# Autodesk Inventor assembly: Assembly_Cube_Kinematic_Mirrormount_Thorlabs_45_PRO_v3
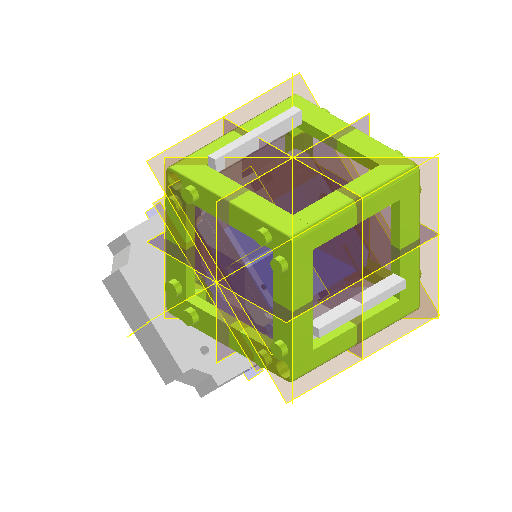
[picture p0: Inventor's stored thumbnail of the model, 512x512]
Saved by Autodesk Inventor 2022 (Build 260153000, 153)
## iProperties
Created: 2021-11-15
Part Number: Assembly_Cube_Kinematic_Mirrormount_Thorlabs_45_PRO_v3
Document SubType Name: Assembly
Designer: diederichbenedict
Author: diederichbenedict
## Documents named in this file (7)
- C:\Users\UC2\Documents\GitHub\openUC2-Hackathon-openOCTRemote\INVENTOR\Assembly_Cube_Kinematic_Mirrormount_Thorlabs_45_PRO_v3.iam
- C:\Users\UC2\Documents\GitHub\openUC2-Hackathon-openOCTRemote\INVENTOR\Assembly_Cube_empty_IM_v3.iam
- C:\Users\UC2\Documents\GitHub\openUC2-Hackathon-openOCTRemote\INVENTOR\00_Thorlabs_PF10-03-P01-Step.ipt
- C:\Users\UC2\Documents\GitHub\openUC2-Hackathon-openOCTRemote\INVENTOR\20_Cube_Insert_Kinematic_Mirror_90_pro_v3.ipt
- C:\Users\UC2\Documents\GitHub\openUC2-Hackathon-openOCTRemote\INVENTOR\20_Cube_Insert_Kinematic_Mirrormount_90_pro_v3.ipt
- C:\Users\UC2\Documents\GitHub\openUC2-Hackathon-openOCTRemote\INVENTOR\20_Cube_Insert_Kinematic_Mirror_45_pro_v3.ipt
- C:\Users\UC2\Documents\GitHub\openUC2-Hackathon-openOCTRemote\INVENTOR\20_Cube_Insert_Kinematic_KES400AMount_90_pro_v3.ipt
## Components (6 placed, 6 different names)
1. Assembly_Cube_empty_IM_v3:1 [sub-assembly] — Passend:8, Passend:9, Passend:10, Fluchtend:1, Fluchtend:2
2. 20_Cube_Insert_Kinematic_Mirrormount_90_pro_v3:1 — Passend:8, Passend:9, Passend:10, Passend:11
3. 20_Cube_Insert_Kinematic_Mirror_90_pro_v3:1 — Passend:11, Winkel:1
4. 00_Thorlabs_PF10-03-P01-Step:1 — Einfügen:1
5. 20_Cube_Insert_Kinematic_Mirror_45_pro_v3:1 — Fluchtend:1, Fluchtend:2, Winkel:1, Passend:12, Winkel:2, Passend:13
6. 20_Cube_Insert_Kinematic_KES400AMount_90_pro_v3:1 — Passend:12, Winkel:2, Passend:13, Einfügen:1
## Relationships (11: Mate 6, Flush 2, Angle 2, Insert 1)
- Passend:8 [Mate]: Assembly_Cube_empty_IM_v3:1 ↔ 20_Cube_Insert_Kinematic_Mirrormount_90_pro_v3:1
- Passend:9 [Mate]: Assembly_Cube_empty_IM_v3:1 ↔ 20_Cube_Insert_Kinematic_Mirrormount_90_pro_v3:1
- Passend:10 [Mate]: Assembly_Cube_empty_IM_v3:1 ↔ 20_Cube_Insert_Kinematic_Mirrormount_90_pro_v3:1
- Fluchtend:1 [Flush]: Assembly_Cube_empty_IM_v3:1 ↔ 20_Cube_Insert_Kinematic_Mirror_45_pro_v3:1
- Fluchtend:2 [Flush]: Assembly_Cube_empty_IM_v3:1 ↔ 20_Cube_Insert_Kinematic_Mirror_45_pro_v3:1
- Passend:11 [Mate]: 20_Cube_Insert_Kinematic_Mirrormount_90_pro_v3:1 ↔ 20_Cube_Insert_Kinematic_Mirror_90_pro_v3:1
- Winkel:1 [Angle] (0 deg): 20_Cube_Insert_Kinematic_Mirror_90_pro_v3:1 ↔ 20_Cube_Insert_Kinematic_Mirror_45_pro_v3:1
- Passend:12 [Mate]: 20_Cube_Insert_Kinematic_Mirror_45_pro_v3:1 ↔ 20_Cube_Insert_Kinematic_KES400AMount_90_pro_v3:1
- Winkel:2 [Angle] (0 deg): 20_Cube_Insert_Kinematic_Mirror_45_pro_v3:1 ↔ 20_Cube_Insert_Kinematic_KES400AMount_90_pro_v3:1
- Passend:13 [Mate] (2 mm): 20_Cube_Insert_Kinematic_Mirror_45_pro_v3:1 ↔ 20_Cube_Insert_Kinematic_KES400AMount_90_pro_v3:1
- Einfügen:1 [Insert]: 00_Thorlabs_PF10-03-P01-Step:1 ↔ 20_Cube_Insert_Kinematic_KES400AMount_90_pro_v3:1
